# Autodesk Inventor assembly: Assembly2
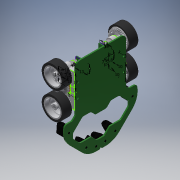
[picture p0: Inventor's stored thumbnail of the model, 180x180]
Saved by Autodesk Inventor 2018 (Build 220112000, 112)
## iProperties
Created: 2017-05-26
Part Number: Assembly2
Material: Ogólny
Document SubType Name: Assembly
Designer: Karol
Author: Karol
## Documents named in this file (6)
- D:\Git\MicromouseDixi\hardware\models\Dixi.iam
- D:\Git\MicromouseDixi\hardware\models\mainpcb.ipt
- D:\Git\MicromouseDixi\hardware\models\led_mount.ipt
- D:\Git\MicromouseDixi\hardware\models\encoder.iam
- D:\Git\MicromouseDixi\hardware\models\driveRight.iam
- D:\Git\MicromouseDixi\hardware\models\driveLeft.iam
## Components (11 placed, 5 different names)
1. mainpcb:1 — Mate:1, Mate:2, Sztywne:1, Sztywne:2, Obrotowe:1, Sztywne:3
2. led_mount:1
3. led_mount:2
4. led_mount:3
5. led_mount:4
6. led_mount:5
7. led_mount:6
8. encoder:1 [sub-assembly] — Sztywne:2
9. encoder:2 [sub-assembly] — Sztywne:1
10. driveLeft:1 [sub-assembly] — Obrotowe:1
11. driveRight:1 [sub-assembly] — Sztywne:3
## Relationships (6: WeldJoint 3, Mate 2, RevoluteJoint 1)
- Mate:1: mainpcb:1
- Mate:2: mainpcb:1
- Sztywne:1 [WeldJoint]: mainpcb:1 ↔ encoder:2
- Sztywne:2 [WeldJoint]: mainpcb:1 ↔ encoder:1
- Obrotowe:1 [RevoluteJoint]: mainpcb:1 ↔ driveLeft:1
- Sztywne:3 [WeldJoint]: mainpcb:1 ↔ driveRight:1
